# Autodesk Inventor assembly: funnel
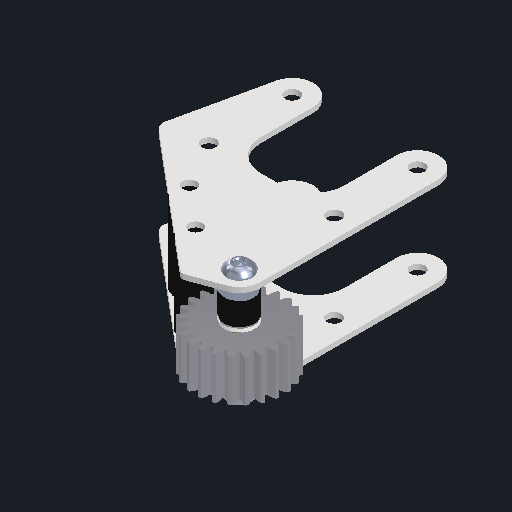
[picture p0: Inventor's stored thumbnail of the model, 512x512]
Saved by Autodesk Inventor 2025 (Build 290162000, 162)
## iProperties
Created: 2024-10-12
Part Number: funnel
Document SubType Name: Assembly
Designer: Averey Ku
Author: Averey Ku
## Documents named in this file (15)
- D:\vex_robotics_high_stakes\hardware\cad\bots\high_stakes_v2\chassis_v2\drivebay\funnel.iam
- D:\vex_robotics_high_stakes\hardware\cad\bots\high_stakes_v2\chassis_v2\drivebay\custom_parts\funel_gusset.ipt
- D:\vex_robotics_high_stakes\hardware\cad\robpros_cad_lib\Motion\Gears\HS Gear\HS 24T Gear, Circle.iam
- D:\vex_robotics_high_stakes\hardware\cad\robpros_cad_lib\Motion\Gears\HS Gear.iam
- D:\vex_robotics_high_stakes\hardware\cad\robpros_cad_lib\Motion\Spacers\Spacer Nylon .375 OD\NSpacer .375 OD x .500.ipt
- D:\vex_robotics_high_stakes\hardware\cad\robpros_cad_lib\Motion\Spacers\Spacer Nylon .375 OD.ipt
- D:\vex_robotics_high_stakes\hardware\cad\robpros_cad_lib\Structure\Hardware\Screw Steel - Star\SScrew Star Smooth 1.250.ipt
- D:\vex_robotics_high_stakes\hardware\cad\robpros_cad_lib\Structure\Hardware\Screw Steel - Star.ipt
- D:\vex_robotics_high_stakes\hardware\cad\robpros_cad_lib\Motion\Spacers\Washer Teflon\TWasher .375 OD x .04000.ipt
- D:\vex_robotics_high_stakes\hardware\cad\robpros_cad_lib\Motion\Spacers\Washer Teflon.ipt
- D:\vex_robotics_high_stakes\hardware\cad\robpros_cad_lib\Structure\Hardware\Nut Keps.ipt
- D:\vex_robotics_high_stakes\hardware\cad\robpros_cad_lib\Structure\Hardware\Nut Thin Nylock.ipt
- D:\vex_robotics_high_stakes\hardware\cad\robpros_cad_lib\Motion\Spacers\Spacer Nylon .375 OD\NSpacer .375 OD x .250.ipt
- D:\vex_robotics_high_stakes\hardware\cad\robpros_cad_lib\Motion\Spacers\Washer Steel\SWasher .375 OD x .015625.ipt
- D:\vex_robotics_high_stakes\hardware\cad\robpros_cad_lib\Motion\Spacers\Washer Steel.ipt
## Components (14 placed, 9 different names)
1. funel_gusset:1 — Insert:10, Insert:15
2. HS 24T Gear, Circle:1 [sub-assembly] — Insert:8
3. funel_gusset:2 — Insert:6, Mate:1, Mate:2, Insert:9, Insert:11
4. NSpacer .375 OD x .500:1 — Insert:6
5. NSpacer .375 OD x .500:2
6. NSpacer .375 OD x .500:3 — Mate:1
7. NSpacer .375 OD x .500:4
8. TWasher .375 OD x .04000:1 — Insert:8, Insert:9
9. Nut Keps:1 — Insert:10, Insert:14
10. Nut Thin Nylock:1 — Insert:11
11. NSpacer .375 OD x .250:5 — Insert:12, Insert:14
12. TWasher .375 OD x .04000:2 — Insert:13
13. SWasher .375 OD x .015625:1 — Insert:12, Insert:13
14. SScrew Star Smooth 1.250:1 — Insert:15
## Relationships (15: Insert 13, Mate 2)
- [Insert]: NSpacer .375 OD x .500:1 ↔ NSpacer .375 OD x .500:2
- [Insert]: funel_gusset:1 ↔ NSpacer .375 OD x .500:2
- [Insert]: NSpacer .375 OD x .500:3 ↔ NSpacer .375 OD x .500:4
- [Insert]: funel_gusset:1 ↔ NSpacer .375 OD x .500:4
- Insert:6: funel_gusset:2 ↔ NSpacer .375 OD x .500:1
- Mate:1: funel_gusset:2 ↔ NSpacer .375 OD x .500:3
- Mate:2: funel_gusset:2
- Insert:8: HS 24T Gear, Circle:1 ↔ TWasher .375 OD x .04000:1
- Insert:9: funel_gusset:2 ↔ TWasher .375 OD x .04000:1
- Insert:10: funel_gusset:1 ↔ Nut Keps:1
- Insert:11: funel_gusset:2 ↔ Nut Thin Nylock:1
- Insert:12: NSpacer .375 OD x .250:5 ↔ SWasher .375 OD x .015625:1
- Insert:13: TWasher .375 OD x .04000:2 ↔ SWasher .375 OD x .015625:1
- Insert:14: Nut Keps:1 ↔ NSpacer .375 OD x .250:5
- Insert:15: funel_gusset:1 ↔ SScrew Star Smooth 1.250:1
## Named parameters: d42_d40 = 0 mm
